# Autodesk Inventor assembly: ArmProto
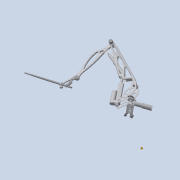
[picture p0: Inventor's stored thumbnail of the model, 180x180]
Saved by Autodesk Inventor 2020.4 (Build 244396010, 396A)
## iProperties
Created: 2020-03-24
Part Number: ArmProto
Document SubType Name: Assembly
Designer: valer
Mass: 4853.13 g
Surface Area: 3141.52 cm^2
Volume: 1403.99 cm^3
Density: 3.45667 g/cm^3
Author: valer
## Documents named in this file (25)
- C:\Users\Val\Desktop\drummingrobot\src\parts\ArmProto.iam
- C:\Users\Val\Desktop\drummingrobot\src\parts\UpperArm.ipt
- C:\Users\Val\Desktop\drummingrobot\src\parts\UpperArmBracket.ipt
- C:\Users\Val\Desktop\drummingrobot\src\parts\Forearm.ipt
- C:\Users\Val\Desktop\drummingrobot\src\parts\external\Drumstick.ipt
- C:\Users\Val\Desktop\drummingrobot\src\parts\external\ForearmShaftCollar.ipt
- C:\Users\Val\Desktop\drummingrobot\src\parts\external\ArmSolenoid.ipt
- C:\Users\Val\Desktop\drummingrobot\src\parts\external\UpperArmActuatorBody.ipt
- C:\Users\Val\Desktop\drummingrobot\src\parts\external\UpperArmActuatorShaft.ipt
- C:\Users\Val\Desktop\drummingrobot\src\parts\external\ForearmActuatorBody.ipt
- C:\Users\Val\Desktop\drummingrobot\src\parts\external\ForearmActuatorShaft.ipt
- C:\Users\Val\Desktop\drummingrobot\src\parts\ForearmActuatorConnector.ipt
- C:\Users\Val\Desktop\drummingrobot\src\parts\SolenoidBracket.ipt
- C:\Users\Val\Desktop\drummingrobot\src\parts\external\ShoulderServo.ipt
- C:\Users\Val\Desktop\drummingrobot\src\parts\UpperArmBracketBase.ipt
- C:\Users\Val\Desktop\drummingrobot\src\parts\external\ShoulderMiterGear.ipt
- C:\Users\Val\Desktop\drummingrobot\src\parts\external\ShoulderServoShaft.ipt
- C:\Users\Val\Desktop\drummingrobot\src\parts\external\ServoShaft.ipt
- C:\Users\Val\Desktop\drummingrobot\src\parts\external\ShoulderMotorMount.ipt
- C:\Users\Val\Desktop\drummingrobot\src\parts\external\PatternSpacer.ipt
- C:\Users\Val\Desktop\JT30.ipt
- C:\Users\Val\Desktop\drummingrobot\src\parts\external\Shoulder6mmDShaftHub-545578.ipt
- C:\Users\Val\Downloads\1123-0043-0072\1123-0043-0072.ipt
- C:\Users\Val\Downloads\1106-0010-0080\1106-0010-0080.ipt
- C:\Users\Val\Downloads\1103-0005-0040\1103-0005-0040.ipt
## Components (34 placed, 23 different names)
1. Drumstick:1 — Mate:79, Flush:3
2. ShaftCollar1/2:1 — Mate:79, Flush:3, Mate:236, Flush:18
3. ArmSolenoid:1 — Mate:290, Mate:291
4. UpperArmActuatorBody:1 — Mate:266, Mate:287
5. Forearm:1 — Flush:17, Mate:227, Mate:236, Flush:18, Mate:288, Mate:289, Mate:348
6. UpperArmActuatorShaft:2 — Mate:238, Flush:20, Mate:266
7. ForearmActuatorBody:1 — Mate:231, Mate:232, Mate:234, Flush:19
8. ForearmActuatorShaft:3 — Flush:17, Mate:231, Mate:232, Mate:342, Mate:344, Mate:345, Mate:346, Angle:13
9. UpperArm:3 — Mate:227, Mate:234, Mate:238, Flush:19, Flush:20, Mate:364, Mate:365, Mate:367, Mate:368, Mate:369, Mate:370
10. ForearmActuatorConnector:1 — Mate:345, Mate:346, Mate:347, Mate:348, Angle:13
11. ForearmActuatorConnector:2 — Mate:342, Mate:344, Mate:347
12. UpperArmBracket:5 — Mate:376, Mate:378, Mate:379
13. UpperArmBracket:6 — Mate:287, Mate:367, Mate:368, Mate:377, Mate:380, Mate:381
14. SolenoidBracket:1 — Mate:288, Mate:289, Mate:290, Mate:291
15. ShoulderServo:1 — Mate:301, Mate:302, Mate:340
16. ShoulderMiterGear:1 — Mate:303, Mate:317
17. ShoulderServoShaft:1 — Mate:301, Mate:302, Mate:303, Mate:316
18. ShoulderMiterGear:2 — Angle:12, Mate:318
19. ShoulderServoShaft:2 — Mate:319, Mate:320, Mate:374
20. ShoulderMotorMount:1 — Mate:316, Angle:12, Flush:24, Flush:26, Mate:340
21. ShoulderMotorMount:2 — Flush:25, Mate:319, Flush:26, Mate:321, Mate:322
22. PatternSpacer:1 — Mate:320, Mate:321, Mate:322, Mate:375
23. ShoulderMotorMount:3 — Mate:382, Mate:383, Mate:384, Mate:385, Angle:14, Mate:386, Mate:387, Angle:15, Mate:388, Mate:389, Angle:16
24. JT30:2 — Mate:364, Mate:365
25. JT30:3 — Mate:369, Mate:370
26. UpperArmBracketBase:1 — Mate:371, Mate:372, Mate:373, Mate:376, Mate:377, Mate:378, Mate:379, Mate:380, Mate:381
27. Shoulder6mmDShaftHub-545578:1 — Mate:371, Mate:372, Mate:373, Mate:374, Mate:375
28. 1123-0043-0072:1 — Mate:390, Mate:391, Mate:392
29. 1106-0010-0080:1 — Mate:382, Mate:383, Mate:390, Mate:392, Mate:393
30. 1106-0010-0080:2 — Mate:384, Mate:385, Angle:14, Mate:394, Mate:395
31. 1106-0010-0080:3 — Mate:388, Mate:389, Angle:16, Mate:396, Mate:398
32. 1106-0010-0080:4 — Mate:386, Mate:387, Angle:15, Mate:391, Mate:397
33. 1103-0005-0040:1 — Mate:393, Mate:394, Mate:395
34. 1103-0005-0040:2 — Mate:396, Mate:397, Mate:398
## Relationships (77: Mate 64, Flush 8, Angle 5)
- Mate:79: Drumstick:1 ↔ ShaftCollar1/2:1
- Flush:3 (304.8 mm): Drumstick:1 ↔ ShaftCollar1/2:1
- Flush:17: Forearm:1 ↔ ForearmActuatorShaft:3
- Mate:227: Forearm:1 ↔ UpperArm:3
- Mate:231: ForearmActuatorBody:1 ↔ ForearmActuatorShaft:3
- Mate:232: ForearmActuatorBody:1 ↔ ForearmActuatorShaft:3
- Mate:234: ForearmActuatorBody:1 ↔ UpperArm:3
- Mate:236: ShaftCollar1/2:1 ↔ Forearm:1
- Flush:18 (12.7 mm): ShaftCollar1/2:1 ↔ Forearm:1
- Mate:238: UpperArmActuatorShaft:2 ↔ UpperArm:3
- Flush:19: ForearmActuatorBody:1 ↔ UpperArm:3
- Flush:20: UpperArmActuatorShaft:2 ↔ UpperArm:3
- Mate:266: UpperArmActuatorBody:1 ↔ UpperArmActuatorShaft:2
- Mate:287: UpperArmActuatorBody:1 ↔ UpperArmBracket:6
- Mate:288: Forearm:1 ↔ SolenoidBracket:1
- Mate:289: Forearm:1 ↔ SolenoidBracket:1
- Mate:290: ArmSolenoid:1 ↔ SolenoidBracket:1
- Mate:291: ArmSolenoid:1 ↔ SolenoidBracket:1
- Mate:301: ShoulderServo:1 ↔ ShoulderServoShaft:1
- Mate:302: ShoulderServo:1 ↔ ShoulderServoShaft:1
- Mate:303: ShoulderMiterGear:1 ↔ ShoulderServoShaft:1
- Mate:316: ShoulderServoShaft:1 ↔ ShoulderMotorMount:1
- Angle:12 (0 deg): ShoulderMiterGear:2 ↔ ShoulderMotorMount:1
- Flush:24: ShoulderMotorMount:1
- Mate:317 (1 mm): ShoulderMiterGear:1
- Mate:318 (1 mm): ShoulderMiterGear:2
- Flush:25: ShoulderMotorMount:2
- Mate:319: ShoulderServoShaft:2 ↔ ShoulderMotorMount:2
- Flush:26: ShoulderMotorMount:1 ↔ ShoulderMotorMount:2
- Mate:320: ShoulderServoShaft:2 ↔ PatternSpacer:1
- Mate:321: ShoulderMotorMount:2 ↔ PatternSpacer:1
- Mate:322: ShoulderMotorMount:2 ↔ PatternSpacer:1
- Mate:340 (2 mm): ShoulderServo:1 ↔ ShoulderMotorMount:1
- Mate:342: ForearmActuatorShaft:3 ↔ ForearmActuatorConnector:2
- Mate:344: ForearmActuatorShaft:3 ↔ ForearmActuatorConnector:2
- Mate:345: ForearmActuatorShaft:3 ↔ ForearmActuatorConnector:1
- Mate:346: ForearmActuatorShaft:3 ↔ ForearmActuatorConnector:1
- Mate:347: ForearmActuatorConnector:1 ↔ ForearmActuatorConnector:2
- Mate:348: Forearm:1 ↔ ForearmActuatorConnector:1
- Angle:13 (-90 deg): ForearmActuatorShaft:3 ↔ ForearmActuatorConnector:1
- Mate:364: UpperArm:3 ↔ JT30:2
- Mate:365: UpperArm:3 ↔ JT30:2
- Mate:367: UpperArm:3 ↔ UpperArmBracket:6
- Mate:368: UpperArm:3 ↔ UpperArmBracket:6
- Mate:369: UpperArm:3 ↔ JT30:3
- Mate:370: UpperArm:3 ↔ JT30:3
- Mate:371: UpperArmBracketBase:1 ↔ Shoulder6mmDShaftHub-545578:1
- Mate:372: UpperArmBracketBase:1 ↔ Shoulder6mmDShaftHub-545578:1
- Mate:373: UpperArmBracketBase:1 ↔ Shoulder6mmDShaftHub-545578:1
- Mate:374: ShoulderServoShaft:2 ↔ Shoulder6mmDShaftHub-545578:1
- Mate:375: PatternSpacer:1 ↔ Shoulder6mmDShaftHub-545578:1
- Mate:376: UpperArmBracket:5 ↔ UpperArmBracketBase:1
- Mate:377: UpperArmBracket:6 ↔ UpperArmBracketBase:1
- Mate:378: UpperArmBracket:5 ↔ UpperArmBracketBase:1
- Mate:379: UpperArmBracket:5 ↔ UpperArmBracketBase:1
- Mate:380: UpperArmBracket:6 ↔ UpperArmBracketBase:1
- Mate:381: UpperArmBracket:6 ↔ UpperArmBracketBase:1
- Mate:382: ShoulderMotorMount:3 ↔ 1106-0010-0080:1
- Mate:383: ShoulderMotorMount:3 ↔ 1106-0010-0080:1
- Mate:384: ShoulderMotorMount:3 ↔ 1106-0010-0080:2
- Mate:385: ShoulderMotorMount:3 ↔ 1106-0010-0080:2
- Angle:14 (0 deg): ShoulderMotorMount:3 ↔ 1106-0010-0080:2
- Mate:386: ShoulderMotorMount:3 ↔ 1106-0010-0080:4
- Mate:387: ShoulderMotorMount:3 ↔ 1106-0010-0080:4
- Angle:15 (0 deg): ShoulderMotorMount:3 ↔ 1106-0010-0080:4
- Mate:388: ShoulderMotorMount:3 ↔ 1106-0010-0080:3
- Mate:389: ShoulderMotorMount:3 ↔ 1106-0010-0080:3
- Angle:16 (0 deg): ShoulderMotorMount:3 ↔ 1106-0010-0080:3
- Mate:390: 1123-0043-0072:1 ↔ 1106-0010-0080:1
- Mate:391: 1123-0043-0072:1 ↔ 1106-0010-0080:4
- Mate:392: 1123-0043-0072:1 ↔ 1106-0010-0080:1
- Mate:393: 1106-0010-0080:1 ↔ 1103-0005-0040:1
- Mate:394: 1106-0010-0080:2 ↔ 1103-0005-0040:1
- Mate:395: 1106-0010-0080:2 ↔ 1103-0005-0040:1
- Mate:396: 1106-0010-0080:3 ↔ 1103-0005-0040:2
- Mate:397: 1106-0010-0080:4 ↔ 1103-0005-0040:2
- Mate:398: 1106-0010-0080:3 ↔ 1103-0005-0040:2
